# Autodesk Inventor assembly: FullAssembly
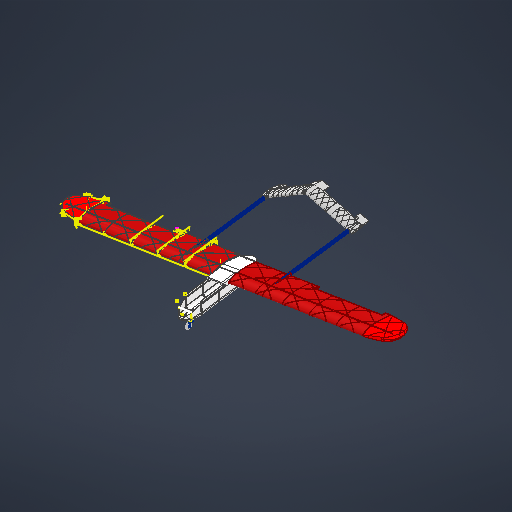
[picture p0: Inventor's stored thumbnail of the model, 512x512]
Saved by Autodesk Inventor 2026.1 (Build 301233000, 233)
## iProperties
Created: 2026-03-02
Part Number: FullAssembly
Document SubType Name: Assembly
Designer: mateo
Author: mateo
## Documents named in this file (9)
- C:\GitHub\Senior-Design-UAV\Elytra CAD\Assembly\FullAssembly.iam
- C:\GitHub\Senior-Design-UAV\Elytra CAD\Fueselage.ipt
- C:\GitHub\Senior-Design-UAV\Elytra CAD\WingRight.ipt
- C:\GitHub\Senior-Design-UAV\Elytra CAD\WingLeft.ipt
- C:\GitHub\Senior-Design-UAV\Elytra CAD\20x20 Extrusions\20x20x2900ExtrudedAluminum.ipt
- C:\GitHub\Senior-Design-UAV\Elytra CAD\Tail.ipt
- C:\GitHub\Senior-Design-UAV\Elytra CAD\20x20 Extrusions\20x20x800ExtrudedAluminum.ipt
- C:\GitHub\Senior-Design-UAV\Elytra CAD\Landing Gear\front landing gear assembly.iam
- C:\GitHub\Senior-Design-UAV\Elytra CAD\Landing Gear\back Landing gear assembly.iam
## Components (9 placed, 8 different names)
1. Fueselage:1 — Mate:10, Mate:11, Mate:12, Mate:13, Mate:14, Mate:16, Mate:18, Mate:20
2. WingRight:1 — Mate:20
3. WingLeft:1 — Mate:18, Mate:19
4. 20x20x2900ExtrudedAluminum:1 — Mate:11, Mate:12, Mate:13, Flush:1, Mate:15, Flush:2, Mate:17
5. Tail:1 — Mate:10, Mate:21
6. 20x20x800ExtrudedAluminum:1 — Mate:14, Flush:1, Mate:15, Mate:19
7. 20x20x800ExtrudedAluminum:2 — Mate:16, Flush:2, Mate:17, Mate:21
8. front landing gear assembly:1 [sub-assembly]
9. back Landing gear assembly:1 [sub-assembly]
## Relationships (14: Mate 12, Flush 2)
- Mate:10: Fueselage:1 ↔ Tail:1
- Mate:11: Fueselage:1 ↔ 20x20x2900ExtrudedAluminum:1
- Mate:12: Fueselage:1 ↔ 20x20x2900ExtrudedAluminum:1
- Mate:13: Fueselage:1 ↔ 20x20x2900ExtrudedAluminum:1
- Mate:14 (381 mm): Fueselage:1 ↔ 20x20x800ExtrudedAluminum:1
- Flush:1: 20x20x2900ExtrudedAluminum:1 ↔ 20x20x800ExtrudedAluminum:1
- Mate:15: 20x20x2900ExtrudedAluminum:1 ↔ 20x20x800ExtrudedAluminum:1
- Mate:16 (381 mm): Fueselage:1 ↔ 20x20x800ExtrudedAluminum:2
- Flush:2: 20x20x2900ExtrudedAluminum:1 ↔ 20x20x800ExtrudedAluminum:2
- Mate:17: 20x20x2900ExtrudedAluminum:1 ↔ 20x20x800ExtrudedAluminum:2
- Mate:18: Fueselage:1 ↔ WingLeft:1
- Mate:19: WingLeft:1 ↔ 20x20x800ExtrudedAluminum:1
- Mate:20: Fueselage:1 ↔ WingRight:1
- Mate:21: Tail:1 ↔ 20x20x800ExtrudedAluminum:2
